# Autodesk Inventor assembly: nc_nhk17
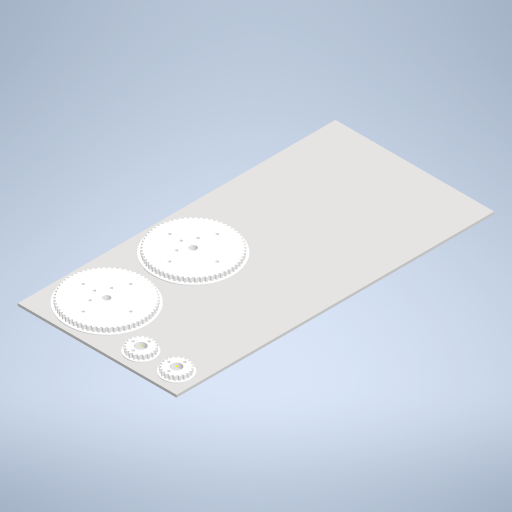
[picture p0: Inventor's stored thumbnail of the model, 512x512]
Saved by Autodesk Inventor 2023 (Build 270158000, 158)
## iProperties
Created: 2022-04-26
Part Number: nc_nhk17
Document SubType Name: Assembly
Designer: yuta
Author: yuta
## Documents named in this file (4)
- C:\Users\yuta\Documents\NHK\nc_nhk17.iam
- C:\Users\yuta\Documents\NHK\旧\NC.port.ipt
- C:\Users\yuta\Documents\NHK\射出_プーリ_歯数60.ipt
- C:\Users\yuta\Documents\NHK\射出_プーリ_歯数20.ipt
## Components (5 placed, 3 different names)
1. NC.port:1 — メイト:1, メイト:2, メイト:3, メイト:4, メイト:5, メイト:6, メイト:7, メイト:8, メイト:9, メイト:10, メイト:11, メイト:12
2. 射出_プーリ_歯数60:1 — メイト:1, メイト:2, メイト:3
3. 射出_プーリ_歯数60:2 — メイト:4, メイト:5, メイト:6
4. 射出_プーリ_歯数20:1 — メイト:7, メイト:9, メイト:10
5. 射出_プーリ_歯数20:2 — メイト:8, メイト:11, メイト:12
## Relationships (12: Mate 12)
- メイト:1 [Mate]: NC.port:1 ↔ 射出_プーリ_歯数60:1
- メイト:2 [Mate] (-56 mm): NC.port:1 ↔ 射出_プーリ_歯数60:1
- メイト:3 [Mate] (-56 mm): NC.port:1 ↔ 射出_プーリ_歯数60:1
- メイト:4 [Mate]: NC.port:1 ↔ 射出_プーリ_歯数60:2
- メイト:5 [Mate] (-56 mm): NC.port:1 ↔ 射出_プーリ_歯数60:2
- メイト:6 [Mate] (-165 mm): NC.port:1 ↔ 射出_プーリ_歯数60:2
- メイト:7 [Mate]: NC.port:1 ↔ 射出_プーリ_歯数20:1
- メイト:8 [Mate]: NC.port:1 ↔ 射出_プーリ_歯数20:2
- メイト:9 [Mate] (-25 mm): NC.port:1 ↔ 射出_プーリ_歯数20:1
- メイト:10 [Mate] (-130 mm): NC.port:1 ↔ 射出_プーリ_歯数20:1
- メイト:11 [Mate] (-25 mm): NC.port:1 ↔ 射出_プーリ_歯数20:2
- メイト:12 [Mate] (-25 mm): NC.port:1 ↔ 射出_プーリ_歯数20:2
